# Autodesk Inventor assembly: MotorRight
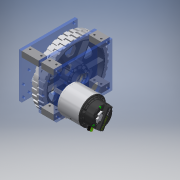
[picture p0: Inventor's stored thumbnail of the model, 180x180]
Saved by Autodesk Inventor 2019 (Build 230136000, 136)
## iProperties
Created: 2020-03-02
Part Number: MotorRight
Document SubType Name: Assembly
Designer: james
Author: james
## Documents named in this file (6)
- F:\JimsRobot\FIRSTRobots\Design\TornadoPlatypus\MotorRight.iam
- F:\JimsRobot\FIRSTRobots\Design\TornadoPlatypus\InsideMotorPlate.ipt
- F:\JimsRobot\FIRSTRobots\Design\Library\CTR\Falcon\217-6515 20191025.iam
- F:\JimsRobot\FIRSTRobots\Design\TornadoPlatypus\MotorSpacerBlock.ipt
- F:\JimsRobot\FIRSTRobots\Design\Library\AndyMark\6 HiGrip Asm Rev II.iam
- F:\JimsRobot\FIRSTRobots\Design\TornadoPlatypus\MotorSpacerBlock2.ipt
## Components (10 placed, 5 different names)
1. InsideMotorPlate:1 — Mate:1, Mate:2, Mate:3, Mate:4, Mate:5, Mate:6, Mate:7, Mate:8, Flush:1, Mate:9, Flush:2, Mate:10, Flush:3, Mate:11, Flush:4
2. 217-6515 20191025:1 [sub-assembly] — Mate:1, Mate:2, Mate:3
3. MotorSpacerBlock:1 — Mate:7, Mate:9, Flush:2
4. MotorSpacerBlock:2 — Mate:4, Mate:11, Flush:4
5. MotorSpacerBlock:3 — Mate:6, Mate:8, Flush:1, Mate:14
6. MotorSpacerBlock:4 — Mate:5, Mate:10, Flush:3, Mate:12, Mate:13
7. InsideMotorPlate:2 — Mate:12, Mate:13, Mate:14, Mate:15, Mate:16, Mate:17, Mate:18, Flush:5, Mate:21
8. 6 HiGrip Asm Rev II:1 [sub-assembly] — Mate:15, Mate:16
9. MotorSpacerBlock2:1 — Mate:17, Mate:18, Flush:5, Mate:19, Mate:20
10. InsideMotorPlate:3 — Mate:19, Mate:20, Mate:21
## Relationships (26: Mate 21, Flush 5)
- Mate:1: InsideMotorPlate:1 ↔ 217-6515 20191025:1
- Mate:2: InsideMotorPlate:1 ↔ 217-6515 20191025:1
- Mate:3: InsideMotorPlate:1 ↔ 217-6515 20191025:1
- Mate:4: InsideMotorPlate:1 ↔ MotorSpacerBlock:2
- Mate:5: InsideMotorPlate:1 ↔ MotorSpacerBlock:4
- Mate:6: InsideMotorPlate:1 ↔ MotorSpacerBlock:3
- Mate:7: InsideMotorPlate:1 ↔ MotorSpacerBlock:1
- Mate:8: InsideMotorPlate:1 ↔ MotorSpacerBlock:3
- Flush:1: InsideMotorPlate:1 ↔ MotorSpacerBlock:3
- Mate:9: InsideMotorPlate:1 ↔ MotorSpacerBlock:1
- Flush:2: InsideMotorPlate:1 ↔ MotorSpacerBlock:1
- Mate:10: InsideMotorPlate:1 ↔ MotorSpacerBlock:4
- Flush:3: InsideMotorPlate:1 ↔ MotorSpacerBlock:4
- Mate:11: InsideMotorPlate:1 ↔ MotorSpacerBlock:2
- Flush:4: InsideMotorPlate:1 ↔ MotorSpacerBlock:2
- Mate:12: MotorSpacerBlock:4 ↔ InsideMotorPlate:2
- Mate:13: MotorSpacerBlock:4 ↔ InsideMotorPlate:2
- Mate:14: MotorSpacerBlock:3 ↔ InsideMotorPlate:2
- Mate:15: InsideMotorPlate:2 ↔ 6 HiGrip Asm Rev II:1
- Mate:16: InsideMotorPlate:2 ↔ 6 HiGrip Asm Rev II:1
- Mate:17: InsideMotorPlate:2 ↔ MotorSpacerBlock2:1
- Mate:18: InsideMotorPlate:2 ↔ MotorSpacerBlock2:1
- Flush:5: InsideMotorPlate:2 ↔ MotorSpacerBlock2:1
- Mate:19: MotorSpacerBlock2:1 ↔ InsideMotorPlate:3
- Mate:20: MotorSpacerBlock2:1 ↔ InsideMotorPlate:3
- Mate:21: InsideMotorPlate:2 ↔ InsideMotorPlate:3
